# Autodesk Inventor assembly: TEST SCREW ARM
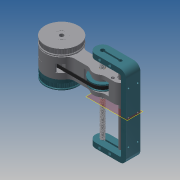
[picture p0: Inventor's stored thumbnail of the model, 180x180]
Saved by Autodesk Inventor 2013 (Build 170138000, 138)
## iProperties
Created: 2017-04-04
Part Number: TEST SCREW ARM
Document SubType Name: Assembly
Designer: employee
Author: employee
## Documents named in this file (15)
- C:\Users\employee\Desktop\SCARA\TEST SCREW ARM.iam
- C:\Users\employee\Desktop\SCARA\SCREW BOTTOM ARM.ipt
- C:\Users\employee\Desktop\SCARA\SCREW TOP ARM.ipt
- C:\Users\employee\Desktop\SCARA\screw nut.iam
- C:\Users\employee\Desktop\SCARA\lm6luu.ipt
- C:\Users\employee\Desktop\SCARA\distal drive pulley.ipt
- C:\Users\employee\Desktop\SCARA\M3x35.ipt
- C:\Users\employee\Desktop\SCARA\M3x30.ipt
- C:\Users\employee\Desktop\SCARA\M8 LEAD SCREW.ipt
- C:\Users\employee\Desktop\SCARA\SCREW slide frame.ipt
- C:\Users\employee\Desktop\SCARA\rod.ipt
- C:\Users\employee\Desktop\SCARA\608 bearing.ipt
- C:\Users\employee\Desktop\SCARA\washer.ipt
- C:\Users\employee\Desktop\SCARA\Z belt.ipt
- C:\Users\employee\Desktop\SCARA\SCREW Z IDLER.ipt
## Components (25 placed, 14 different names)
1. SCREW BOTTOM ARM:1 — Mate:1, Insert:11, Insert:16, Mate:6
2. SCREW TOP ARM:1 — Mate:1, Insert:3, Insert:4, Insert:5, Insert:6, Insert:7, Insert:8, Insert:9, Insert:10, Mate:2, Insert:11, Mate:3, Mate:5, Insert:20
3. lm6luu:1 — Insert:3
4. distal drive pulley:1 — Insert:10, Mate:2, Mate:3, Insert:12, Insert:13, Insert:14, Insert:15, Insert:19
5. M3x35:1 — Insert:7
6. M3x35:2 — Insert:6
7. M3x35:3 — Insert:5
8. M3x35:4 — Insert:4
9. M3x35:5 — Insert:9
10. M3x35:6 — Insert:8
11. M3x30:1 — Insert:12
12. M3x30:2 — Insert:14
13. M3x30:3 — Insert:15
14. M3x30:4 — Insert:13
15. screw nut:1 [sub-assembly] — Insert:16, Mate:4, Rotation/Translation:1, Insert:22
16. M8 LEAD SCREW:1 — Mate:4, Rotation/Translation:1, Insert:17
17. SCREW slide frame:1 — Insert:17, Insert:18
18. rod:1 — Insert:18, Mate:5
19. 608 bearing:1 — Insert:19
20. 608 bearing:2 — Insert:20, Insert:21
21. washer:1 — Insert:21, Insert:25
22. Z belt:1 — Insert:22, Mate:6
23. SCREW Z IDLER:1 — Insert:23, Insert:24
24. 608 bearing:3 — Insert:23
25. 608 bearing:4 — Insert:24, Insert:25
## Relationships (30: Insert 23, Mate 6, RelateRotateTranslate 1)
- Mate:1: SCREW BOTTOM ARM:1 ↔ SCREW TOP ARM:1
- Insert:3: SCREW TOP ARM:1 ↔ lm6luu:1
- Insert:4: SCREW TOP ARM:1 ↔ M3x35:4
- Insert:5: SCREW TOP ARM:1 ↔ M3x35:3
- Insert:6: SCREW TOP ARM:1 ↔ M3x35:2
- Insert:7: SCREW TOP ARM:1 ↔ M3x35:1
- Insert:8: SCREW TOP ARM:1 ↔ M3x35:6
- Insert:9: SCREW TOP ARM:1 ↔ M3x35:5
- Insert:10: SCREW TOP ARM:1 ↔ distal drive pulley:1
- Mate:2: SCREW TOP ARM:1 ↔ distal drive pulley:1
- Insert:11: SCREW BOTTOM ARM:1 ↔ SCREW TOP ARM:1
- Mate:3: SCREW TOP ARM:1 ↔ distal drive pulley:1
- Insert:12: distal drive pulley:1 ↔ M3x30:1
- Insert:13: distal drive pulley:1 ↔ M3x30:4
- Insert:14: distal drive pulley:1 ↔ M3x30:2
- Insert:15: distal drive pulley:1 ↔ M3x30:3
- Insert:16: SCREW BOTTOM ARM:1 ↔ screw nut:1
- Mate:4: screw nut:1 ↔ M8 LEAD SCREW:1
- Rotation/Translation:1 [RelateRotateTranslate] (1.5 mm): screw nut:1 ↔ M8 LEAD SCREW:1
- Insert:17 (5 mm): M8 LEAD SCREW:1 ↔ SCREW slide frame:1
- Insert:18 (5 mm): SCREW slide frame:1 ↔ rod:1
- Mate:5: SCREW TOP ARM:1 ↔ rod:1
- Insert:19: distal drive pulley:1 ↔ 608 bearing:1
- Insert:20: SCREW TOP ARM:1 ↔ 608 bearing:2
- Insert:21: 608 bearing:2 ↔ washer:1
- Insert:22 (1 mm): screw nut:1 ↔ Z belt:1
- Mate:6: SCREW BOTTOM ARM:1 ↔ Z belt:1
- Insert:23: SCREW Z IDLER:1 ↔ 608 bearing:3
- Insert:24: SCREW Z IDLER:1 ↔ 608 bearing:4
- Insert:25: washer:1 ↔ 608 bearing:4
